# Autodesk Inventor assembly: 組合檔
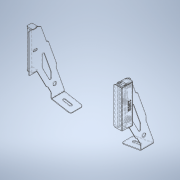
[picture p0: Inventor's stored thumbnail of the model, 180x180]
Saved by Autodesk Inventor 2020 (Build 240168000, 168)
## iProperties
Created: 2015-11-28
Part Number: 組合檔
Document SubType Name: Assembly
Designer: 設計製圖
Author: 設計製圖
## Documents named in this file (13)
- D:\資料庫\設計-3D Project\【May club 】\得利卡-車頂燈架\模型、圖面\短-車頂燈架-組合(#11.02)-總組合.iam
- D:\資料庫\設計-3D Project\材料庫\【螺絲】\止付螺絲\止付螺絲-M8-20.ipt
- D:\資料庫\設計-3D Project\【May club 】\得利卡-車頂燈架\模型、圖面\車身圖.ipt
- D:\資料庫\設計-3D Project\【May club 】\得利卡-車頂燈架\模型、圖面\得利卡-車頂導水槽.ipt
- D:\資料庫\設計-3D Project\材料庫\【螺絲】\外六角螺絲\白鐵-外六角  M6-20.ipt
- D:\資料庫\設計-3D Project\材料庫\【華司】\白鐵-平面華司-7-16-2t.ipt
- D:\資料庫\設計-3D Project\材料庫\【華司】\彈簧華司\白鐵-彈簧華司-6.ipt
- D:\資料庫\設計-3D Project\【May club 】\得利卡-車頂燈架\模型、圖面\短-車頂燈架-組合(#11.02)-生產圖面_21.11.26\製程筆記\封邊條 ( 平光黑 ) - 130L.ipt
- D:\資料庫\設計-3D Project\【May club 】\得利卡-車頂燈架\模型、圖面\短-車頂燈架-組合(#11.02)-生產圖面_21.11.26\製程筆記\背膠海綿eva 6T -  15W x 125L.ipt
- D:\資料庫\設計-3D Project\【May club 】\得利卡-車頂燈架\模型、圖面\短-車頂燈架-組合(#11.02)-生產圖面_21.11.26\製程筆記\背膠海綿eva 3T -  25W x 125L.ipt
- D:\資料庫\設計-3D Project\【May club 】\得利卡-車頂燈架\模型、圖面\短-車頂燈架-組合(#11.02)-生產圖面_21.11.26\製程筆記\背膠海綿eva 3T -  10W x 125L.ipt
- D:\資料庫\設計-3D Project\【May club 】\得利卡-車頂燈架\模型、圖面\短-車頂燈架-組合(#11.02)- 組合件1.iam
- D:\資料庫\設計-3D Project\【May club 】\得利卡-車頂燈架\模型、圖面\短-車頂燈架-組合(#11.02)- 組合件2.iam
## Components (13 placed, 12 different names)
1. 短-車頂燈架-組合(#11.02)- 組合件1:1 [sub-assembly] — 貼合:66, 貼合:67, 貼合:68, 貼合:69, 齊平:15, 貼合:70, 齊平:16, 貼合:73
2. 短-車頂燈架-組合(#11.02)- 組合件2:1 [sub-assembly] — 貼合:63, 貼合:64, 貼合:65, 齊平:13, 齊平:14, 貼合:71, 貼合:72, 齊平:16, 貼合:74
3. 得利卡-車頂導水槽:1
4. 車身圖:1
5. 背膠海綿eva 6T -  15W x 125L:1 — 貼合:66, 貼合:67, 貼合:68
6. 背膠海綿eva 3T -  25W x 125L:1 — 貼合:62, 貼合:63, 貼合:64, 齊平:14
7. 背膠海綿eva 3T -  10W x 125L:1 — 貼合:62, 貼合:65, 齊平:13
8. 白鐵-彈簧華司-6:1 — 貼合:49, 貼合:51, 貼合:52
9. 白鐵-平面華司-7-16-2t:1 — 貼合:48, 貼合:51
10. 白鐵-外六角  M6-20:1 — 貼合:48, 貼合:49, 貼合:52, 貼合:74
11. 封邊條 ( 平光黑 ) - 130L:1 — 貼合:69, 齊平:15, 貼合:70
12. 止付螺絲-M8-20:1 — 齊平:12, 貼合:71, 貼合:73
13. 止付螺絲-M8-20:2 — 齊平:12, 貼合:72
## Relationships (22: Mate 17, Flush 5)
- 齊平:12 [Flush]: 止付螺絲-M8-20:1 ↔ 止付螺絲-M8-20:2
- 貼合:48 [Mate]: 白鐵-平面華司-7-16-2t:1 ↔ 白鐵-外六角  M6-20:1
- 貼合:49 [Mate]: 白鐵-彈簧華司-6:1 ↔ 白鐵-外六角  M6-20:1
- 貼合:51 [Mate]: 白鐵-彈簧華司-6:1 ↔ 白鐵-平面華司-7-16-2t:1
- 貼合:52 [Mate]: 白鐵-彈簧華司-6:1 ↔ 白鐵-外六角  M6-20:1
- 貼合:62 [Mate]: 背膠海綿eva 3T -  25W x 125L:1 ↔ 背膠海綿eva 3T -  10W x 125L:1
- 貼合:63 [Mate]: 短-車頂燈架-組合(#11.02)- 組合件2:1 ↔ 背膠海綿eva 3T -  25W x 125L:1
- 貼合:64 [Mate]: 短-車頂燈架-組合(#11.02)- 組合件2:1 ↔ 背膠海綿eva 3T -  25W x 125L:1
- 貼合:65 [Mate]: 短-車頂燈架-組合(#11.02)- 組合件2:1 ↔ 背膠海綿eva 3T -  10W x 125L:1
- 齊平:13 [Flush]: 短-車頂燈架-組合(#11.02)- 組合件2:1 ↔ 背膠海綿eva 3T -  10W x 125L:1
- 齊平:14 [Flush]: 短-車頂燈架-組合(#11.02)- 組合件2:1 ↔ 背膠海綿eva 3T -  25W x 125L:1
- 貼合:66 [Mate]: 短-車頂燈架-組合(#11.02)- 組合件1:1 ↔ 背膠海綿eva 6T -  15W x 125L:1
- 貼合:67 [Mate]: 短-車頂燈架-組合(#11.02)- 組合件1:1 ↔ 背膠海綿eva 6T -  15W x 125L:1
- 貼合:68 [Mate]: 短-車頂燈架-組合(#11.02)- 組合件1:1 ↔ 背膠海綿eva 6T -  15W x 125L:1
- 貼合:69 [Mate]: 短-車頂燈架-組合(#11.02)- 組合件1:1 ↔ 封邊條 ( 平光黑 ) - 130L:1
- 齊平:15 [Flush]: 短-車頂燈架-組合(#11.02)- 組合件1:1 ↔ 封邊條 ( 平光黑 ) - 130L:1
- 貼合:70 [Mate]: 短-車頂燈架-組合(#11.02)- 組合件1:1 ↔ 封邊條 ( 平光黑 ) - 130L:1
- 貼合:71 [Mate]: 短-車頂燈架-組合(#11.02)- 組合件2:1 ↔ 止付螺絲-M8-20:1
- 貼合:72 [Mate]: 短-車頂燈架-組合(#11.02)- 組合件2:1 ↔ 止付螺絲-M8-20:2
- 齊平:16 [Flush]: 短-車頂燈架-組合(#11.02)- 組合件1:1 ↔ 短-車頂燈架-組合(#11.02)- 組合件2:1
- 貼合:73 [Mate]: 短-車頂燈架-組合(#11.02)- 組合件1:1 ↔ 止付螺絲-M8-20:1
- 貼合:74 [Mate]: 短-車頂燈架-組合(#11.02)- 組合件2:1 ↔ 白鐵-外六角  M6-20:1
